# Autodesk Inventor assembly: Montagem Ventuinha
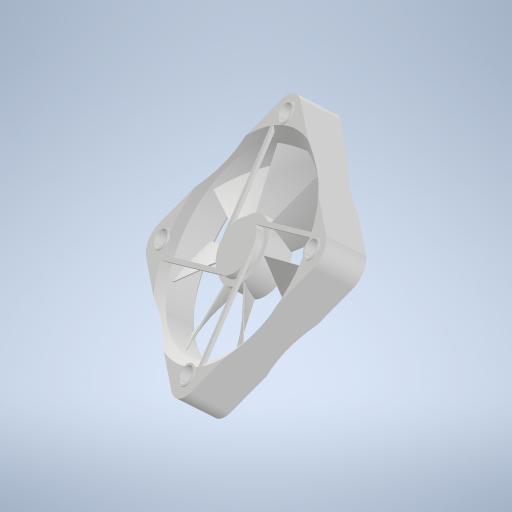
[picture p0: Inventor's stored thumbnail of the model, 512x512]
Saved by Autodesk Inventor 2023.2 (Build 272271000, 271)
## iProperties
Created: 2022-12-19
Part Number: Montagem Ventuinha
Document SubType Name: Assembly
Designer: coqui
Author: coqui
## Documents named in this file (3)
- D:\Felipe Coquito\OneDrive\Documents\Inventor\Inventor - curso\Montagem\Montagem Ventuinha.iam
- D:\Felipe Coquito\OneDrive\Documents\Inventor\Inventor - curso\Ventoinha\Ventoinha.ipt
- D:\Felipe Coquito\OneDrive\Documents\Inventor\Inventor - curso\Ventoinha\Suporte da Ventoinha.ipt
## Components (2 placed, 2 different names)
1. Ventoinha:1 — Mate:1, Mate:2
2. Suporte da Ventoinha:1 — Mate:1, Mate:2
## Relationships (2: Mate 2)
- Mate:1: Ventoinha:1 ↔ Suporte da Ventoinha:1
- Mate:2: Ventoinha:1 ↔ Suporte da Ventoinha:1
